# Autodesk Inventor assembly: NikkonTubelensAssembly
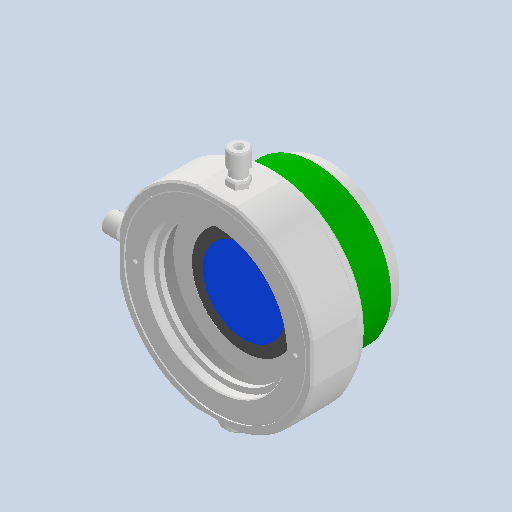
[picture p0: Inventor's stored thumbnail of the model, 512x512]
Saved by Autodesk Inventor 2026.1 (Build 301233000, 233)
## iProperties
Created: 2019-08-07
Part Number: NikkonTubelensAssembly
Document SubType Name: Assembly
Designer: Julian
Author: Julian
## Documents named in this file (4)
- C:\Users\user\Desktop\setup_inventor_2025\LightPath\lens\NikkonTubelensAssembly.iam
- C:\Users\user\Desktop\setup_inventor_2025\LightPath\lens\SM2LensXYmount.ipt
- C:\Users\user\Desktop\setup_inventor_2025\LightPath\lens\SM2exM38in.ipt
- C:\Users\user\Desktop\setup_inventor_2025\LightPath\lens\NikkonTubelens.ipt
## Components (3 placed, 3 different names)
1. SM2LensXYmount:1 — Passend:2, Passend:3
2. SM2exM38in:1 — Passend:1, Passend:2, Fluchtend:1, Passend:3
3. NikkonTubelens:1 — Passend:1, Fluchtend:1
## Relationships (4: Mate 3, Flush 1)
- Passend:1 [Mate]: SM2exM38in:1 ↔ NikkonTubelens:1
- Passend:2 [Mate]: SM2LensXYmount:1 ↔ SM2exM38in:1
- Fluchtend:1 [Flush]: SM2exM38in:1 ↔ NikkonTubelens:1
- Passend:3 [Mate] (5 mm): SM2LensXYmount:1 ↔ SM2exM38in:1
